# Autodesk Inventor assembly: recuperation
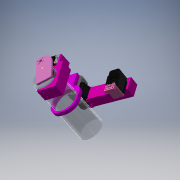
[picture p0: Inventor's stored thumbnail of the model, 180x180]
Saved by Autodesk Inventor 2017 (Build 210142000, 142)
## iProperties
Created: 2018-03-31
Part Number: recuperation
Document SubType Name: Assembly
Designer: franc
Mass: 403.773 g
Surface Area: 1652.88 cm^2
Volume: 403.773 cm^3
Density: 1 g/cm^3
Author: franc
## Documents named in this file (10)
- C:\Users\franc\Desktop\EsialRobotik\Mecanique\2018\robot\traitement-eau\recuperation.iam
- C:\Users\franc\Desktop\EsialRobotik\Mecanique\2018\robot\traitement-eau\cylindre-stockage.ipt
- C:\Users\franc\Desktop\EsialRobotik\Mecanique\composants\AX12\AX12.iam
- C:\Users\franc\Desktop\EsialRobotik\Mecanique\2018\robot\traitement-eau\trappe.ipt
- C:\Users\franc\Desktop\EsialRobotik\Mecanique\composants\AX12\F3.ipt
- C:\Users\franc\Desktop\EsialRobotik\Mecanique\2018\robot\traitement-eau\support-trappe.ipt
- C:\Users\franc\Desktop\EsialRobotik\Mecanique\composants\AX12\F2.ipt
- C:\Users\franc\Desktop\EsialRobotik\Mecanique\2018\robot\traitement-eau\rotation-recuperation.ipt
- C:\Users\franc\Desktop\EsialRobotik\Mecanique\2018\robot\traitement-eau\bras.ipt
- C:\Users\franc\Desktop\EsialRobotik\Mecanique\2018\robot\traitement-eau\fixation-bras.ipt
## Components (11 placed, 9 different names)
1. cylindre-stockage:1 — Affleurement:1, Tangente:7, Tangente:8, Tangente:9, Affleurement:3, Placage:22
2. AX12:1 [sub-assembly] — Affleurement:1, Tangente:5, Tangente:6, Placage:5, Placage:6, Placage:7, Placage:8, Tangente:7, Tangente:8
3. trappe:1 — Tangente:5, Tangente:6, Placage:5
4. F3:1 — Placage:6, Placage:7, Placage:8, Placage:9, Affleurement:2, Placage:10
5. support-trappe:1 — Placage:9, Affleurement:2, Placage:10, Affleurement:4
6. F2:1 — Tangente:9, Affleurement:3, Affleurement:4, Placage:14, Affleurement:5, Placage:25, Placage:26, Placage:27
7. rotation-recuperation:1 — Placage:14, Affleurement:5, Placage:22
8. bras:1 — Placage:28, Placage:29, Placage:30, Placage:31, Placage:32, Placage:33
9. AX12:2 [sub-assembly] — Placage:19, Placage:20, Placage:21, Placage:31, Placage:32, Placage:33
10. fixation-bras:1 — Placage:19, Placage:20, Placage:21
11. AX12:3 [sub-assembly] — Placage:25, Placage:26, Placage:27, Placage:28, Placage:29, Placage:30
## Relationships (30: Mate 20, Flush 5, Tangent 5)
- Affleurement:1 [Flush]: cylindre-stockage:1 ↔ AX12:1
- Tangente:5: AX12:1 ↔ trappe:1
- Tangente:6: AX12:1 ↔ trappe:1
- Placage:5 [Mate]: AX12:1 ↔ trappe:1
- Placage:6 [Mate]: AX12:1 ↔ F3:1
- Placage:7 [Mate]: AX12:1 ↔ F3:1
- Placage:8 [Mate]: AX12:1 ↔ F3:1
- Tangente:7 (1 mm): cylindre-stockage:1 ↔ AX12:1
- Tangente:8: cylindre-stockage:1 ↔ AX12:1
- Placage:9 [Mate]: F3:1 ↔ support-trappe:1
- Affleurement:2 [Flush]: F3:1 ↔ support-trappe:1
- Placage:10 [Mate]: F3:1 ↔ support-trappe:1
- Tangente:9 (1 mm): cylindre-stockage:1 ↔ F2:1
- Affleurement:3 [Flush] (87.5 mm): cylindre-stockage:1 ↔ F2:1
- Affleurement:4 [Flush] (25.5 mm): support-trappe:1 ↔ F2:1
- Placage:14 [Mate]: F2:1 ↔ rotation-recuperation:1
- Affleurement:5 [Flush]: F2:1 ↔ rotation-recuperation:1
- Placage:19 [Mate]: AX12:2 ↔ fixation-bras:1
- Placage:20 [Mate]: AX12:2 ↔ fixation-bras:1
- Placage:21 [Mate]: AX12:2 ↔ fixation-bras:1
- Placage:22 [Mate]: cylindre-stockage:1 ↔ rotation-recuperation:1
- Placage:25 [Mate]: F2:1 ↔ AX12:3
- Placage:26 [Mate]: F2:1 ↔ AX12:3
- Placage:27 [Mate]: F2:1 ↔ AX12:3
- Placage:28 [Mate]: bras:1 ↔ AX12:3
- Placage:29 [Mate]: bras:1 ↔ AX12:3
- Placage:30 [Mate]: bras:1 ↔ AX12:3
- Placage:31 [Mate]: bras:1 ↔ AX12:2
- Placage:32 [Mate]: bras:1 ↔ AX12:2
- Placage:33 [Mate]: bras:1 ↔ AX12:2
